# Autodesk Inventor assembly: SCARA_montagem
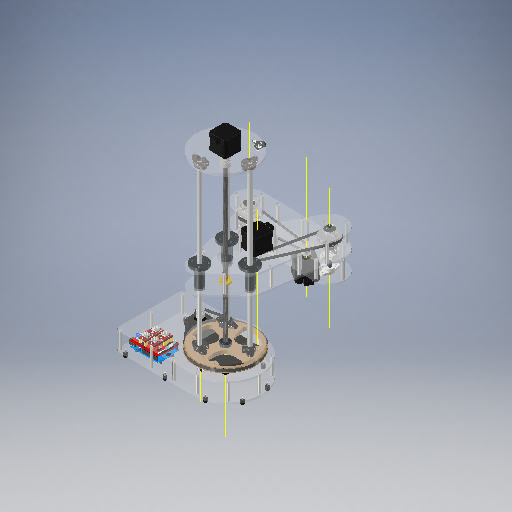
[picture p0: Inventor's stored thumbnail of the model, 512x512]
Saved by Autodesk Inventor 2025.1 (Build 291241020, 241B)
## iProperties
Created: 2025-05-02
Part Number: SCARA_montagem
Document SubType Name: Assembly
Designer: Nelson
Author: Nelson
## Documents named in this file (4)
- C:\Users\tiago\Documents\Inventor\SCRA\SCARA_montagem.iam
- C:\Users\tiago\Documents\Inventor\SCRA\Base-Rotation.iam
- C:\Users\tiago\Documents\Inventor\SCRA\Elo_sup.iam
- C:\Users\tiago\Documents\Inventor\SCRA\F_TOPO.iam
## Components (3 placed, 3 different names)
1. Base-Rotation:1 [sub-assembly] — Flush:1, Mate:2, Mate:3, Mate:4, Mate:5, Mate:6, Mate:7
2. Elo_sup:1 [sub-assembly] — Mate:1, Mate:4, Rotation/Translation:1
3. F_TOPO:1 [sub-assembly] — Mate:1, Mate:2, Mate:3, Mate:5, Rotation/Translation:1
## Relationships (9: Mate 7, Flush 1, RelateRotateTranslate 1)
- Flush:1: Base-Rotation:1
- Mate:1: Elo_sup:1 ↔ F_TOPO:1
- Mate:2: Base-Rotation:1 ↔ F_TOPO:1
- Mate:3: Base-Rotation:1 ↔ F_TOPO:1
- Mate:4: Base-Rotation:1 ↔ Elo_sup:1
- Mate:5: Base-Rotation:1 ↔ F_TOPO:1
- Mate:6: Base-Rotation:1
- Mate:7: Base-Rotation:1
- Rotation/Translation:1 [RelateRotateTranslate] (25.133 mm): Elo_sup:1 ↔ F_TOPO:1
